# Autodesk Inventor assembly: BancEcoShell
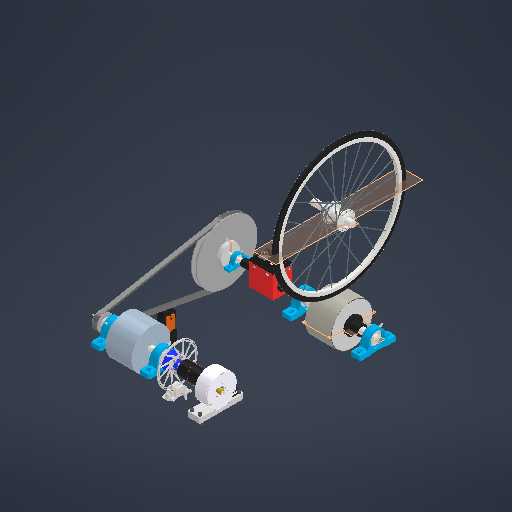
[picture p0: Inventor's stored thumbnail of the model, 512x512]
Saved by Autodesk Inventor 2026.2 (Build 302298010, 298A)
## iProperties
Created: 2026-03-31
Part Number: BancEcoShell
Document SubType Name: Assembly
Designer: romai
Author: romai
## Documents named in this file (29)
- D:\Downloads\LogicielMaster\Inventor\Enssemble\BancEcoShell\BancEcoShell.iam
- D:\Downloads\LogicielMaster\Inventor\Pièces\Couplemètre.ipt
- D:\Downloads\LogicielMaster\Inventor\Pièces\Rouleau.ipt
- C:\Users\romai\Documents\Inventor\Content Center Files\R2026\fr-FR\ISO 1207(2)\ISO 1207 - M2 x 3.ipt
- D:\Downloads\LogicielMaster\Inventor\Enssemble\BancEcoShell\ArbreRoue1.ipt
- D:\Downloads\LogicielMaster\Inventor\Enssemble\BancEcoShell\ArbreCouplemètre1.ipt
- D:\Downloads\LogicielMaster\Inventor\Pièces\RoueVelo.ipt
- D:\Downloads\LogicielMaster\Inventor\Enssemble\BancEcoShell\ArbrePrimaire2.ipt
- D:\Downloads\LogicielMaster\Inventor\Enssemble\BancEcoShell\ArbreRoue2.ipt
- D:\Downloads\LogicielMaster\Inventor\Enssemble\BancEcoShell\ArbreSecondaire2.ipt
- D:\Downloads\LogicielMaster\Inventor\Enssemble\BancEcoShell\BancEcoShell\Design Accelerator\Transmission par courroie trapézoïdale2.iam
- D:\Downloads\LogicielMaster\Inventor\Pièces\Frein.ipt
- D:\Downloads\LogicielMaster\Inventor\Enssemble\BancEcoShell\ArbrePoulie1.ipt
- D:\Downloads\LogicielMaster\Inventor\Enssemble\BancEcoShell\SupportArbre.ipt
- D:\Downloads\LogicielMaster\Inventor\Enssemble\BancEcoShell\Palier.ipt
- D:\Downloads\LogicielMaster\Inventor\Enssemble\BancEcoShell\Flasque.ipt
- D:\Downloads\LogicielMaster\Inventor\Enssemble\BancEcoShell\Masse.ipt
- D:\Downloads\LogicielMaster\Inventor\Enssemble\BancEcoShell\Douille2517.ipt
- D:\Downloads\LogicielMaster\Inventor\Enssemble\BancEcoShell\Douille1008.ipt
- D:\Downloads\LogicielMaster\Inventor\Enssemble\BancEcoShell\SupportTendeur.ipt
- D:\Downloads\LogicielMaster\Inventor\Enssemble\BancEcoShell\RouleauTendeur.ipt
- C:\Users\romai\Documents\Inventor\Content Center Files\R2026\fr-FR\ISO 1207(2)\ISO 1207 - M5 x 6.ipt
- D:\Downloads\LogicielMaster\Inventor\Enssemble\BancEcoShell\Befestigung bremsscheibe.ipt
- D:\Downloads\LogicielMaster\Inventor\Enssemble\BancEcoShell\DisqueFrein.ipt
- C:\Users\romai\Documents\Inventor\Content Center Files\R2026\fr-FR\ISO 4762(2)\ISO 4762 - M6 x 10ISO.ipt
- D:\Downloads\LogicielMaster\Inventor\Enssemble\BancEcoShell\Accouplement12-25.ipt
- D:\Downloads\LogicielMaster\Inventor\Enssemble\BancEcoShell\Accouplement10-10.ipt
- D:\Downloads\LogicielMaster\Inventor\Enssemble\BancEcoShell\Palier15.ipt
- D:\Downloads\LogicielMaster\Inventor\Enssemble\BancEcoShell\F005 - Brake Calliper.iam
## Components (44 placed, 28 different names)
1. Couplemètre:1 — Placage:1, Placage:2, Placage:3, Affleurement:5, Placage:10, Placage:11, Placage:15, Placage:16
2. ArbreCouplemètre:1 — Placage:3, Affleurement:5, Placage:14, Angle:4, Placage:82, Angle:27, Placage:84, Placage:85, Placage:86, Angle:28, Angle:29, Placage:87, Placage:88
3. ArbrePrimaire:2 — Placage:85, Placage:86, Angle:28, Placage:89, Placage:94, Placage:95, Affleurement:12, Angle:30
4. Rouleau:1 — Rotation:1, Placage:9, Placage:26, Placage:27, Angle:8, Angle:9, Placage:91, Placage:93, Angle:30
5. RoueVelo:1 — Rotation:1, Placage:9, Placage:10, Placage:11, Placage:12, Affleurement:1, Angle:3
6. ArbreRoue:1 — Placage:12, Affleurement:1, Angle:3, Angle:20
7. ArbreSecondaire:1 — Placage:15, Placage:16, Angle:6, Angle:7, Placage:22, Placage:40, Angle:17, Placage:42, Placage:43, Affleurement:7, Placage:49, Placage:61, Angle:25, Placage:78, Placage:81, Angle:26
8. ArbrePoulie:1 — Placage:14, Angle:4, Placage:18, Angle:5, Affleurement:11, Placage:82, Placage:83, Placage:96, Placage:97
9. Transmission par courroie trapézoïdale:1 [sub-assembly] — Placage:18, Angle:5, Angle:6, Placage:41, Affleurement:7, Angle:21, Affleurement:8, Placage:47, Placage:48, Angle:22, Affleurement:9, Placage:49, Tangente:1, Affleurement:10, Affleurement:11, Placage:98, Placage:99
10. Frein:1 — Placage:19, Placage:20, Placage:21, Placage:22, Angle:16, Placage:79
11. ArbreFrein:1 — Placage:19, Placage:20, Placage:21, Angle:7, Placage:80
12. SupportArbre:1 — Placage:26, Angle:8, Placage:31, Placage:36, Angle:10, Placage:92
13. SupportArbre:2 — Placage:27, Angle:9, Placage:32, Placage:37, Angle:11, Placage:90, Placage:94
14. Palier:1 — Placage:31, Angle:12, Placage:95
15. Palier:2 — Placage:32, Angle:13, Placage:89, Affleurement:12
16. Flasque:1 — Placage:36, Angle:10, Placage:92, Placage:93
17. Flasque:2 — Placage:37, Angle:11, Placage:90, Placage:91
18. Masse:1 — Placage:40, Placage:41, Angle:17, Placage:44, Placage:45
19. Palier:5 — Placage:42, Angle:19, Placage:44, Placage:62
20. Palier:6 — Placage:43, Angle:18, Placage:45
21. Douille2517:1 — Angle:21, Affleurement:8, Placage:47
22. Douille1008:1 — Placage:48, Angle:22, Affleurement:9
23. SupportTendeur:1 — Placage:50, Placage:51, Placage:52, Placage:53, Placage:54, Placage:55
24. RouleauTendeur:1 — Placage:50, Placage:51, Tangente:1, Placage:56
25. ISO 1207 M5 x 6:1 — Placage:52, Placage:53
26. ISO 1207 M5 x 6:2 — Placage:54, Placage:55
27. Befestigung bremsscheibe:1 — Placage:61, Placage:62, Angle:25, Placage:63, Placage:64, Placage:65, Placage:66, Placage:68, Placage:70, Placage:72, Placage:74, Placage:76
28. DisqueFrein:1 — Placage:63, Placage:64, Placage:65, Placage:67, Placage:69, Placage:71, Placage:73, Placage:75, Placage:77
29. ISO 4762 M6 x 10:1 — Placage:66, Placage:67
30. ISO 4762 M6 x 10:2 — Placage:68, Placage:69
31. ISO 4762 M6 x 10:3 — Placage:70, Placage:71
32. ISO 4762 M6 x 10:4 — Placage:72, Placage:73
33. ISO 4762 M6 x 10:5 — Placage:74, Placage:75
34. ISO 4762 M6 x 10:6 — Placage:76, Placage:77
35. Accouplement12-25:1 — Placage:78, Placage:79, Placage:80, Placage:81, Angle:26
36. Accouplement10-10:1 — Placage:83, Angle:27, Placage:84
37. Accouplement10-10:2 — Angle:29, Placage:87, Placage:88
38. Palier15:1 — Placage:97, Placage:98, Angle:31
39. Palier15:2 — Placage:96, Placage:99, Angle:32
40. F005 - Brake Calliper:1 [sub-assembly]
41. ISO 1207 M2 x 3:1 — Placage:1, Placage:2
42. ISO 1207 M2 x 3:2
43. ISO 1207 M2 x 3:3
44. ISO 1207 M2 x 3:4
## Component patterns: (4 elements, first: ISO 1207 M2 x 3:1)
## Relationships (112: Mate 76, Angle 26, Flush 8, RelateRotation 1, Tangent 1)
- Placage:1 [Mate]: Couplemètre:1 ↔ ISO 1207 M2 x 3:1
- Placage:2 [Mate]: Couplemètre:1 ↔ ISO 1207 M2 x 3:1
- Placage:3 [Mate]: Couplemètre:1 ↔ ArbreCouplemètre:1
- Affleurement:5 [Flush]: Couplemètre:1 ↔ ArbreCouplemètre:1
- Rotation:1 [RelateRotation] (8.25 ul): Rouleau:1 ↔ RoueVelo:1
- Placage:9 [Mate]: Rouleau:1 ↔ RoueVelo:1
- Placage:10 [Mate]: Couplemètre:1 ↔ RoueVelo:1
- Placage:11 [Mate] (278 mm): Couplemètre:1 ↔ RoueVelo:1
- Placage:12 [Mate]: RoueVelo:1 ↔ ArbreRoue:1
- Affleurement:1 [Flush] (-25 mm): RoueVelo:1 ↔ ArbreRoue:1
- Angle:3 (0 deg): RoueVelo:1 ↔ ArbreRoue:1
- Placage:14 [Mate]: ArbreCouplemètre:1 ↔ ArbrePoulie:1
- Angle:4 (0 deg): ArbreCouplemètre:1 ↔ ArbrePoulie:1
- Placage:15 [Mate] (467 mm): Couplemètre:1 ↔ ArbreSecondaire:1
- Placage:16 [Mate] (-57.5 mm): Couplemètre:1 ↔ ArbreSecondaire:1
- Placage:18 [Mate]: ArbrePoulie:1 ↔ Transmission par courroie trapézoïdale:1
- Angle:5 (0 deg): ArbrePoulie:1 ↔ Transmission par courroie trapézoïdale:1
- Angle:6 (0 deg): ArbreSecondaire:1 ↔ Transmission par courroie trapézoïdale:1
- Placage:19 [Mate]: Frein:1 ↔ ArbreFrein:1
- Placage:20 [Mate]: Frein:1 ↔ ArbreFrein:1
- Placage:21 [Mate]: Frein:1 ↔ ArbreFrein:1
- Angle:7 (0 deg): ArbreSecondaire:1 ↔ ArbreFrein:1
- Placage:22 [Mate]: ArbreSecondaire:1 ↔ Frein:1
- Placage:26 [Mate]: Rouleau:1 ↔ SupportArbre:1
- Placage:27 [Mate]: Rouleau:1 ↔ SupportArbre:2
- Angle:8 (0 deg): Rouleau:1 ↔ SupportArbre:1
- Angle:9 (0 deg): Rouleau:1 ↔ SupportArbre:2
- Placage:31 [Mate] (20 mm): SupportArbre:1 ↔ Palier:1
- Placage:32 [Mate] (20 mm): SupportArbre:2 ↔ Palier:2
- Placage:36 [Mate]: SupportArbre:1 ↔ Flasque:1
- Placage:37 [Mate]: SupportArbre:2 ↔ Flasque:2
- Angle:10 (0 deg): SupportArbre:1 ↔ Flasque:1
- Angle:11 (0 deg): SupportArbre:2 ↔ Flasque:2
- Angle:12 (180 deg): Palier:1
- Angle:13 (180 deg): Palier:2
- Angle:16 (180 deg): Frein:1
- Placage:40 [Mate]: ArbreSecondaire:1 ↔ Masse:1
- Placage:41 [Mate] (75 mm): Transmission par courroie trapézoïdale:1 ↔ Masse:1
- Angle:17 (0 deg): ArbreSecondaire:1 ↔ Masse:1
- Placage:42 [Mate]: ArbreSecondaire:1 ↔ Palier:5
- Placage:43 [Mate]: ArbreSecondaire:1 ↔ Palier:6
- Angle:18 (180 deg): Palier:6
- Angle:19 (180 deg): Palier:5
- Placage:44 [Mate] (19 mm): Masse:1 ↔ Palier:5
- Placage:45 [Mate] (19 mm): Masse:1 ↔ Palier:6
- Affleurement:7 [Flush] (-5 mm): ArbreSecondaire:1 ↔ Transmission par courroie trapézoïdale:1
- Angle:20 (-3600 deg): ArbreRoue:1
- Angle:21 (180 deg): Transmission par courroie trapézoïdale:1 ↔ Douille2517:1
- Affleurement:8 [Flush] (-10 mm): Transmission par courroie trapézoïdale:1 ↔ Douille2517:1
- Placage:47 [Mate]: Transmission par courroie trapézoïdale:1 ↔ Douille2517:1
- Placage:48 [Mate]: Transmission par courroie trapézoïdale:1 ↔ Douille1008:1
- Angle:22 (0 deg): Transmission par courroie trapézoïdale:1 ↔ Douille1008:1
- Affleurement:9 [Flush] (-0.15 mm): Transmission par courroie trapézoïdale:1 ↔ Douille1008:1
- Placage:49 [Mate]: ArbreSecondaire:1 ↔ Transmission par courroie trapézoïdale:1
- Placage:50 [Mate]: SupportTendeur:1 ↔ RouleauTendeur:1
- Placage:51 [Mate]: SupportTendeur:1 ↔ RouleauTendeur:1
- Tangente:1: Transmission par courroie trapézoïdale:1 ↔ RouleauTendeur:1
- Placage:52 [Mate]: SupportTendeur:1 ↔ ISO 1207 M5 x 6:1
- Placage:53 [Mate]: SupportTendeur:1 ↔ ISO 1207 M5 x 6:1
- Placage:54 [Mate]: SupportTendeur:1 ↔ ISO 1207 M5 x 6:2
- Placage:55 [Mate]: SupportTendeur:1 ↔ ISO 1207 M5 x 6:2
- Affleurement:10 [Flush] (-11 mm): Transmission par courroie trapézoïdale:1
- Placage:56 [Mate]: RouleauTendeur:1
- Affleurement:11 [Flush] (50 mm): ArbrePoulie:1 ↔ Transmission par courroie trapézoïdale:1
- Placage:61 [Mate]: ArbreSecondaire:1 ↔ Befestigung bremsscheibe:1
- Placage:62 [Mate] (25 mm): Palier:5 ↔ Befestigung bremsscheibe:1
- Angle:25 (0 deg): ArbreSecondaire:1 ↔ Befestigung bremsscheibe:1
- Placage:63 [Mate]: Befestigung bremsscheibe:1 ↔ DisqueFrein:1
- Placage:64 [Mate]: Befestigung bremsscheibe:1 ↔ DisqueFrein:1
- Placage:65 [Mate]: Befestigung bremsscheibe:1 ↔ DisqueFrein:1
- Placage:66 [Mate]: Befestigung bremsscheibe:1 ↔ ISO 4762 M6 x 10:1
- Placage:67 [Mate]: DisqueFrein:1 ↔ ISO 4762 M6 x 10:1
- Placage:68 [Mate]: Befestigung bremsscheibe:1 ↔ ISO 4762 M6 x 10:2
- Placage:69 [Mate]: DisqueFrein:1 ↔ ISO 4762 M6 x 10:2
- Placage:70 [Mate]: Befestigung bremsscheibe:1 ↔ ISO 4762 M6 x 10:3
- Placage:71 [Mate]: DisqueFrein:1 ↔ ISO 4762 M6 x 10:3
- Placage:72 [Mate]: Befestigung bremsscheibe:1 ↔ ISO 4762 M6 x 10:4
- Placage:73 [Mate]: DisqueFrein:1 ↔ ISO 4762 M6 x 10:4
- Placage:74 [Mate]: Befestigung bremsscheibe:1 ↔ ISO 4762 M6 x 10:5
- Placage:75 [Mate]: DisqueFrein:1 ↔ ISO 4762 M6 x 10:5
- Placage:76 [Mate]: Befestigung bremsscheibe:1 ↔ ISO 4762 M6 x 10:6
- Placage:77 [Mate]: DisqueFrein:1 ↔ ISO 4762 M6 x 10:6
- Placage:78 [Mate]: ArbreSecondaire:1 ↔ Accouplement12-25:1
- Placage:79 [Mate]: Frein:1 ↔ Accouplement12-25:1
- Placage:80 [Mate]: ArbreFrein:1 ↔ Accouplement12-25:1
- Placage:81 [Mate]: ArbreSecondaire:1 ↔ Accouplement12-25:1
- Angle:26 (0 deg): ArbreSecondaire:1 ↔ Accouplement12-25:1
- Placage:82 [Mate] (10 mm): ArbreCouplemètre:1 ↔ ArbrePoulie:1
- Placage:83 [Mate]: ArbrePoulie:1 ↔ Accouplement10-10:1
- Angle:27 (180 deg): ArbreCouplemètre:1 ↔ Accouplement10-10:1
- Placage:84 [Mate] (-15 mm): ArbreCouplemètre:1 ↔ Accouplement10-10:1
- Placage:85 [Mate]: ArbreCouplemètre:1 ↔ ArbrePrimaire:2
- Placage:86 [Mate] (15 mm): ArbreCouplemètre:1 ↔ ArbrePrimaire:2
- Angle:28 (0 deg): ArbreCouplemètre:1 ↔ ArbrePrimaire:2
- Angle:29 (0 deg): ArbreCouplemètre:1 ↔ Accouplement10-10:2
- Placage:87 [Mate]: ArbreCouplemètre:1 ↔ Accouplement10-10:2
- Placage:88 [Mate] (-15 mm): ArbreCouplemètre:1 ↔ Accouplement10-10:2
- Placage:89 [Mate]: ArbrePrimaire:2 ↔ Palier:2
- Placage:90 [Mate]: SupportArbre:2 ↔ Flasque:2
- Placage:91 [Mate]: Rouleau:1 ↔ Flasque:2
- Placage:92 [Mate]: SupportArbre:1 ↔ Flasque:1
- Placage:93 [Mate]: Rouleau:1 ↔ Flasque:1
- Placage:94 [Mate]: ArbrePrimaire:2 ↔ SupportArbre:2
- Placage:95 [Mate]: ArbrePrimaire:2 ↔ Palier:1
- Affleurement:12 [Flush] (-10 mm): ArbrePrimaire:2 ↔ Palier:2
- Angle:30 (0 deg): ArbrePrimaire:2 ↔ Rouleau:1
- Placage:96 [Mate]: ArbrePoulie:1 ↔ Palier15:2
- Placage:97 [Mate]: ArbrePoulie:1 ↔ Palier15:1
- Placage:98 [Mate] (25 mm): Transmission par courroie trapézoïdale:1 ↔ Palier15:1
- Placage:99 [Mate] (25 mm): Transmission par courroie trapézoïdale:1 ↔ Palier15:2
- Angle:31 (180 deg): Palier15:1
- Angle:32 (180 deg): Palier15:2
